# Autodesk Inventor assembly: Head
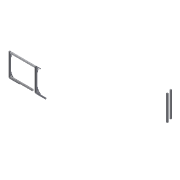
[picture p0: Inventor's stored thumbnail of the model, 180x180]
Saved by Autodesk Inventor 2014 SP1 (Build 180222100, 222)
## iProperties
Created: 2015-02-11
Part Number: Head
Document SubType Name: Assembly
Designer: Simen
Author: Simen
## Documents named in this file (8)
- C:\Users\Simen\Documents\git\Eit\skjellet\Head.iam
- C:\Users\Simen\Documents\git\Eit\skjellet\KHFS5_2020_350.ipt
- C:\Users\Simen\Documents\git\Eit\skjellet\HBL45TS6hbl45ts6.ipt
- C:\Users\Simen\Documents\git\Eit\skjellet\HBL135TS6.iam
- C:\Users\Simen\Documents\git\Eit\skjellet\KHFS5_2020_386.ipt
- C:\Users\Simen\Documents\git\Eit\skjellet\KHFS5_2020_391.ipt
- C:\Users\Simen\Documents\git\Eit\skjellet\KHFS5_2020_247,5.ipt
- C:\Users\Simen\Documents\git\Eit\skjellet\KHFS5_2020_287,5.ipt
## Components (12 placed, 3 different names)
1. HBL45TS6hbl45ts6:1 — Mate:1, Flush:1, Mate:2, Mate:42, Flush:38, Mate:43
2. KHFS5-2020-4000:1 — Mate:1, Flush:1, Mate:2, Mate:6, Flush:5, Mate:7, Mate:30, Flush:23, Flush:24, Mate:40, Flush:36, Flush:37
3. HBL135TS6:1 [sub-assembly] — Mate:6, Flush:5, Mate:7
4. KHFS5-2020-4000:7 — Mate:39, Flush:34, Flush:35
5. HBL45TS6hbl45ts6:2 — Mate:41, Flush:39, Mate:44
6. HBL135TS6:2 [sub-assembly]
7. KHFS5-2020-4000:11 — Mate:30, Flush:23, Flush:24
8. KHFS5-2020-4000:17 — Mate:39, Flush:34, Flush:35, Mate:40, Flush:36, Flush:37
9. KHFS5-2020-4000:18 — Mate:41, Flush:39, Mate:44
10. KHFS5-2020-4000:19 — Mate:42, Flush:38, Mate:43, Flush:40, Mate:45, Flush:41
11. KHFS5-2020-4000:20 — Flush:40, Mate:45, Flush:41
12. KHFS5-2020-4000:21
## Relationships (30: Mate 16, Flush 14)
- Mate:1: HBL45TS6hbl45ts6:1 ↔ KHFS5-2020-4000:1
- Flush:1: HBL45TS6hbl45ts6:1 ↔ KHFS5-2020-4000:1
- Mate:2: HBL45TS6hbl45ts6:1 ↔ KHFS5-2020-4000:1
- Mate:6: KHFS5-2020-4000:1 ↔ HBL135TS6:1
- Flush:5: KHFS5-2020-4000:1 ↔ HBL135TS6:1
- Mate:7: KHFS5-2020-4000:1 ↔ HBL135TS6:1
- [Mate]: KHFS5-2020-4000:7 ↔ HBL45TS6hbl45ts6:2
- [Flush]: KHFS5-2020-4000:7 ↔ HBL45TS6hbl45ts6:2
- [Mate]: KHFS5-2020-4000:7 ↔ HBL45TS6hbl45ts6:2
- [Mate]: KHFS5-2020-4000:7 ↔ HBL135TS6:2
- [Flush]: KHFS5-2020-4000:7 ↔ HBL135TS6:2
- [Mate]: KHFS5-2020-4000:7 ↔ HBL135TS6:2
- Mate:30: KHFS5-2020-4000:1 ↔ KHFS5-2020-4000:11
- Flush:23: KHFS5-2020-4000:1 ↔ KHFS5-2020-4000:11
- Flush:24: KHFS5-2020-4000:1 ↔ KHFS5-2020-4000:11
- Mate:39: KHFS5-2020-4000:7 ↔ KHFS5-2020-4000:17
- Flush:34: KHFS5-2020-4000:7 ↔ KHFS5-2020-4000:17
- Flush:35: KHFS5-2020-4000:7 ↔ KHFS5-2020-4000:17
- Mate:40: KHFS5-2020-4000:1 ↔ KHFS5-2020-4000:17
- Flush:36: KHFS5-2020-4000:1 ↔ KHFS5-2020-4000:17
- Flush:37: KHFS5-2020-4000:1 ↔ KHFS5-2020-4000:17
- Mate:41: HBL45TS6hbl45ts6:2 ↔ KHFS5-2020-4000:18
- Mate:42: HBL45TS6hbl45ts6:1 ↔ KHFS5-2020-4000:19
- Flush:38: HBL45TS6hbl45ts6:1 ↔ KHFS5-2020-4000:19
- Flush:39: HBL45TS6hbl45ts6:2 ↔ KHFS5-2020-4000:18
- Mate:43: HBL45TS6hbl45ts6:1 ↔ KHFS5-2020-4000:19
- Mate:44: HBL45TS6hbl45ts6:2 ↔ KHFS5-2020-4000:18
- Flush:40: KHFS5-2020-4000:19 ↔ KHFS5-2020-4000:20
- Mate:45: KHFS5-2020-4000:19 ↔ KHFS5-2020-4000:20
- Flush:41: KHFS5-2020-4000:19 ↔ KHFS5-2020-4000:20
## Named parameters: d13_d0 = 0 mm, d14_d1 = 0 mm, d15_d2 = 0 mm, d16_d10 = 0 mm, d17_d11 = 0 mm, d18_d12 = 0 mm
